# Autodesk Inventor assembly: GE-17025_ASM_174_ASM
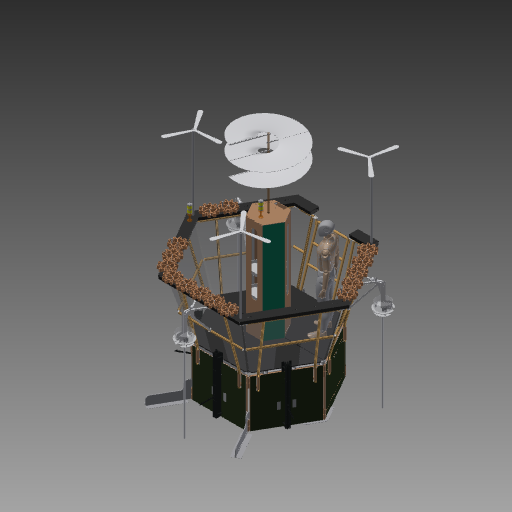
[picture p0: Inventor's stored thumbnail of the model, 512x512]
Saved by Autodesk Inventor 2017.1 (Build 211199000, 199)
## iProperties
Created: 2016-12-16
Part Number: GE-17025_ASM_174_ASM
Document SubType Name: Assembly
Designer: PhillipD
Author: PhillipD
Revision Number: 1LAST_VERSION
## Documents named in this file (25)
- D:\FIRST\FIRST KOP 2017\FRC 2017 Field\Parts\GE-17025_ASM_174_ASM.iam
- D:\FIRST\FIRST KOP 2017\FRC 2017 Field\Parts\GE-17026_ASM_28_ASM.iam
- D:\FIRST\FIRST KOP 2017\FRC 2017 Field\Parts\GE-17033_ASM_16_ASM.iam
- D:\FIRST\FIRST KOP 2017\FRC 2017 Field\Parts\GE-17034_6.ipt
- D:\FIRST\FIRST KOP 2017\FRC 2017 Field\Parts\GE-17044_ASM_20_ASM.iam
- D:\FIRST\FIRST KOP 2017\FRC 2017 Field\Parts\GE-17079_ASM_12_ASM.iam
- D:\FIRST\FIRST KOP 2017\FRC 2017 Field\Parts\AS2_ROPE_6.ipt
- D:\FIRST\FIRST KOP 2017\FRC 2017 Field\Parts\GE-17046_ASM_34_ASM.iam
- D:\FIRST\FIRST KOP 2017\FRC 2017 Field\Parts\GE-17075_ASM_7_ASM.iam
- D:\FIRST\FIRST KOP 2017\FRC 2017 Field\Parts\GE-17085_8.ipt
- D:\FIRST\FIRST KOP 2017\FRC 2017 Field\Parts\GE-17088_ASM_44_ASM.iam
- D:\FIRST\FIRST KOP 2017\FRC 2017 Field\Parts\GE-17092_3.ipt
- D:\FIRST\FIRST KOP 2017\FRC 2017 Field\Parts\GE-17098_14.ipt
- D:\FIRST\FIRST KOP 2017\FRC 2017 Field\Parts\GE-17099_6.ipt
- D:\FIRST\FIRST KOP 2017\FRC 2017 Field\Parts\GE-17069_ASM_14_ASM.iam
- D:\FIRST\FIRST KOP 2017\FRC 2017 Field\Parts\GE-17070_11.ipt
- D:\FIRST\FIRST KOP 2017\FRC 2017 Field\Parts\GE-17071_ASM_15_ASM.iam
- D:\FIRST\FIRST KOP 2017\FRC 2017 Field\Parts\GE-17072_ASM_9_ASM.iam
- D:\FIRST\FIRST KOP 2017\FRC 2017 Field\Parts\GE-17101_ASM_13_ASM.iam
- D:\FIRST\FIRST KOP 2017\FRC 2017 Field\Parts\LIGHT_ASM_ASM_3_ASM.iam
- D:\FIRST\FIRST KOP 2017\FRC 2017 Field\Parts\TOUCHPAD_ASSEMBLY_V3_ASM_ASM_2_ASM.iam
- D:\FIRST\FIRST KOP 2017\FRC 2017 Field\Parts\GE-17025-01_1.ipt
- D:\FIRST\FIRST KOP 2017\FRC 2017 Field\Parts\FUEL_TANK_ASM_1_ASM.iam
- D:\FIRST\FIRST KOP 2017\FRC 2017 Field\Parts\DA_VINCI_PROP_ASM_1_ASM.iam
- D:\FIRST\FIRST KOP 2017\FRC 2017 Field\Parts\JARDE_DUMMY_ASM_3_ASM.iam
## Components (70 placed, 70 different names)
1. GE-17026_ASM_28_ASM_1105 [sub-assembly]
2. GE-17033_ASM_16_ASM_1117 [sub-assembly]
3. GE-17033_ASM_16_ASM_1118 [sub-assembly]
4. GE-17034_6_1119 — Flush:2, Flush:4, Mate:2, Mate:7, Mate:8, Mate:9
5. GE-17034_6_1120 — Flush:3, Flush:5, Flush:8, Flush:9
6. GE-17044_ASM_20_ASM_1130 [sub-assembly] — Tangent:6
7. GE-17044_ASM_20_ASM_1131 [sub-assembly] — Tangent:8
8. GE-17044_ASM_20_ASM_1132 [sub-assembly]
9. GE-17044_ASM_20_ASM_1133 [sub-assembly]
10. GE-17044_ASM_20_ASM_1134 [sub-assembly] — Tangent:7
11. GE-17079_ASM_12_ASM_1151 [sub-assembly]
12. GE-17079_ASM_12_ASM_1152 [sub-assembly] — Mate:10, Mate:11
13. GE-17079_ASM_12_ASM_1153 [sub-assembly]
14. JARDE_DUMMY_ASM_3_ASM_1154 [sub-assembly]
15. AS2_ROPE_6_1155
16. AS2_ROPE_6_1156
17. AS2_ROPE_6_1157
18. GE-17046_ASM_34_ASM_1213 [sub-assembly]
19. GE-17046_ASM_34_ASM_1214 [sub-assembly]
20. GE-17046_ASM_34_ASM_1215 [sub-assembly]
21. GE-17075_ASM_7_ASM_1222 [sub-assembly]
22. GE-17075_ASM_7_ASM_1223 [sub-assembly]
23. GE-17085_8_1224
24. GE-17085_8_1225
25. GE-17085_8_1226
26. GE-17085_8_1227
27. GE-17085_8_1228
28. GE-17085_8_1229
29. GE-17088_ASM_44_ASM_1277 [sub-assembly] — Insert:1, Insert:2, Insert:3, Flush:5, Flush:6, Flush:7, Flush:8, Flush:9, Insert:4, Insert:5, Mate:4, Mate:5, Insert:6, Insert:7, Insert:8, Insert:9, Insert:10, Insert:11, Insert:12, Insert:13, Tangent:3, Insert:14, Insert:15, Insert:16, Insert:17, Insert:18, Tangent:4, Drive Me Gears 1, Tangent:9, Drive Me Gears 2
30. GE-17092_3_1278 — Insert:3
31. GE-17092_3_1279 — Insert:1
32. GE-17092_3_1280 — Insert:2
33. GE-17098_14_1281 — Mate:9, Tangent:8
34. GE-17098_14_1282 — Mate:7, Tangent:6
35. GE-17098_14_1283 — Mate:8, Tangent:7
36. GE-17099_6_1284
37. GE-17099_6_1285
38. GE-17069_ASM_14_ASM_1292 [sub-assembly]
39. GE-17070_11_1293
40. GE-17070_11_1294
41. GE-17071_ASM_15_ASM_1304 [sub-assembly]
42. GE-17072_ASM_9_ASM_1310 [sub-assembly]
43. GE-17101_ASM_13_ASM_1313 [sub-assembly] — Insert:4, Rotation:1, Align Gears 1
44. GE-17101_ASM_13_ASM_1314 [sub-assembly] — Insert:5, Rotation:1, Align Gears 1, Drive Me Gears 1, Tangent:9
45. GE-17101_ASM_13_ASM_1315 [sub-assembly] — Insert:6, Tangent:3, Align Gears 2a, Drive Me Gears 2, Rotation:2
46. GE-17101_ASM_13_ASM_1316 [sub-assembly] — Insert:7, Align Gears 2a, Align Gears 2b, Rotation:2, Rotation:3
47. GE-17101_ASM_13_ASM_1317 [sub-assembly] — Insert:8, Align Gears 2b, Align Gears 2c, Rotation:3, Rotation:4
48. GE-17101_ASM_13_ASM_1318 [sub-assembly] — Insert:9, Align Gears 2d, Align Gears 2c, Rotation:4, Rotation:5
49. GE-17101_ASM_13_ASM_1319 [sub-assembly] — Insert:10, Align Gears 2e, Align Gears 2d, Rotation:5, Rotation:8
50. GE-17101_ASM_13_ASM_1320 [sub-assembly] — Insert:11, Align Gears 2f, Align Gears 2e, Rotation:6, Rotation:8
51. GE-17101_ASM_13_ASM_1321 [sub-assembly] — Insert:12, Align Gears 2g, Align Gears 2f, Rotation:6, Rotation:7
52. GE-17101_ASM_13_ASM_1322 [sub-assembly] — Insert:13, Align Gears 2g, Rotation:7
53. GE-17101_ASM_13_ASM_1323 [sub-assembly] — Insert:14, Tangent:4
54. GE-17101_ASM_13_ASM_1324 [sub-assembly] — Insert:15
55. GE-17101_ASM_13_ASM_1325 [sub-assembly] — Insert:16
56. GE-17101_ASM_13_ASM_1326 [sub-assembly] — Insert:17
57. GE-17101_ASM_13_ASM_1327 [sub-assembly] — Insert:18
58. LIGHT_ASM_ASM_3_ASM_1335 [sub-assembly] — Mate:4, Mate:5
59. LIGHT_ASM_ASM_3_ASM_1336 [sub-assembly]
60. TOUCHPAD_ASSEMBLY_V3_ASM_ASM_2_ASM_1376 [sub-assembly] — Flush:10, Mate:10, Mate:11
61. TOUCHPAD_ASSEMBLY_V3_ASM_ASM_2_ASM_1377 [sub-assembly] — Flush:10
62. TOUCHPAD_ASSEMBLY_V3_ASM_ASM_2_ASM_1378 [sub-assembly]
63. GE-17025-01_1_1379
64. GE-17025-01_1_1380
65. GE-17025-01_1_1381
66. GE-17025-01_1_1382
67. GE-17025-01_1_1383
68. GE-17025-01_1_1384
69. FUEL_TANK_ASM_1_ASM_1416 [sub-assembly] — Mate:1, Flush:1, Flush:2, Flush:3, Flush:4, Mate:2, Flush:6, Flush:7
70. DA_VINCI_PROP_ASM_1_ASM_1424 [sub-assembly] — Mate:1, Flush:1
## Relationships (61: Insert 18, Mate 16, Flush 10, RelateRotation 8, Tangent 6, Angle 3)
- Insert:1: GE-17088_ASM_44_ASM_1277 ↔ GE-17092_3_1279
- Insert:2: GE-17088_ASM_44_ASM_1277 ↔ GE-17092_3_1280
- Insert:3: GE-17088_ASM_44_ASM_1277 ↔ GE-17092_3_1278
- Mate:1: FUEL_TANK_ASM_1_ASM_1416 ↔ DA_VINCI_PROP_ASM_1_ASM_1424
- Flush:1 (-1266.825 mm): FUEL_TANK_ASM_1_ASM_1416 ↔ DA_VINCI_PROP_ASM_1_ASM_1424
- Flush:2 (635 mm): GE-17034_6_1119 ↔ FUEL_TANK_ASM_1_ASM_1416
- Flush:3 (635.0254 mm): GE-17034_6_1120 ↔ FUEL_TANK_ASM_1_ASM_1416
- Flush:4 (635 mm): GE-17034_6_1119 ↔ FUEL_TANK_ASM_1_ASM_1416
- Mate:2: GE-17034_6_1119 ↔ FUEL_TANK_ASM_1_ASM_1416
- Flush:5 (-1107.2876 mm): GE-17034_6_1120 ↔ GE-17088_ASM_44_ASM_1277
- Flush:6 (1015.0602 mm): GE-17088_ASM_44_ASM_1277 ↔ FUEL_TANK_ASM_1_ASM_1416
- Flush:7 (1014.603 mm): GE-17088_ASM_44_ASM_1277 ↔ FUEL_TANK_ASM_1_ASM_1416
- Flush:8 (-1107.2876 mm): GE-17034_6_1120 ↔ GE-17088_ASM_44_ASM_1277
- Flush:9 (-1107.2876 mm): GE-17034_6_1120 ↔ GE-17088_ASM_44_ASM_1277
- Insert:4: GE-17088_ASM_44_ASM_1277 ↔ GE-17101_ASM_13_ASM_1313
- Insert:5: GE-17088_ASM_44_ASM_1277 ↔ GE-17101_ASM_13_ASM_1314
- Rotation:1 [RelateRotation] (1 ul): GE-17101_ASM_13_ASM_1313 ↔ GE-17101_ASM_13_ASM_1314
- Mate:4: GE-17088_ASM_44_ASM_1277 ↔ LIGHT_ASM_ASM_3_ASM_1335
- Mate:5: GE-17088_ASM_44_ASM_1277 ↔ LIGHT_ASM_ASM_3_ASM_1335
- Insert:6: GE-17088_ASM_44_ASM_1277 ↔ GE-17101_ASM_13_ASM_1315
- Insert:7: GE-17088_ASM_44_ASM_1277 ↔ GE-17101_ASM_13_ASM_1316
- Insert:8: GE-17088_ASM_44_ASM_1277 ↔ GE-17101_ASM_13_ASM_1317
- Insert:9: GE-17088_ASM_44_ASM_1277 ↔ GE-17101_ASM_13_ASM_1318
- Insert:10: GE-17088_ASM_44_ASM_1277 ↔ GE-17101_ASM_13_ASM_1319
- Insert:11: GE-17088_ASM_44_ASM_1277 ↔ GE-17101_ASM_13_ASM_1320
- Insert:12: GE-17088_ASM_44_ASM_1277 ↔ GE-17101_ASM_13_ASM_1321
- Insert:13: GE-17088_ASM_44_ASM_1277 ↔ GE-17101_ASM_13_ASM_1322
- Tangent:3: GE-17088_ASM_44_ASM_1277 ↔ GE-17101_ASM_13_ASM_1315
- Insert:14: GE-17088_ASM_44_ASM_1277 ↔ GE-17101_ASM_13_ASM_1323
- Insert:15: GE-17088_ASM_44_ASM_1277 ↔ GE-17101_ASM_13_ASM_1324
- Insert:16: GE-17088_ASM_44_ASM_1277 ↔ GE-17101_ASM_13_ASM_1325
- Insert:17: GE-17088_ASM_44_ASM_1277 ↔ GE-17101_ASM_13_ASM_1326
- Insert:18: GE-17088_ASM_44_ASM_1277 ↔ GE-17101_ASM_13_ASM_1327
- Tangent:4: GE-17088_ASM_44_ASM_1277 ↔ GE-17101_ASM_13_ASM_1323
- Align Gears 1 [Mate]: GE-17101_ASM_13_ASM_1313 ↔ GE-17101_ASM_13_ASM_1314
- Drive Me Gears 1 [Angle] (0 deg): GE-17088_ASM_44_ASM_1277 ↔ GE-17101_ASM_13_ASM_1314
- Mate:7: GE-17034_6_1119 ↔ GE-17098_14_1282
- Tangent:6: GE-17044_ASM_20_ASM_1130 ↔ GE-17098_14_1282
- Mate:8: GE-17034_6_1119 ↔ GE-17098_14_1283
- Tangent:7: GE-17044_ASM_20_ASM_1134 ↔ GE-17098_14_1283
- Mate:9: GE-17034_6_1119 ↔ GE-17098_14_1281
- Tangent:8: GE-17044_ASM_20_ASM_1131 ↔ GE-17098_14_1281
- Flush:10: TOUCHPAD_ASSEMBLY_V3_ASM_ASM_2_ASM_1376 ↔ TOUCHPAD_ASSEMBLY_V3_ASM_ASM_2_ASM_1377
- Mate:10: GE-17079_ASM_12_ASM_1152 ↔ TOUCHPAD_ASSEMBLY_V3_ASM_ASM_2_ASM_1376
- Mate:11: GE-17079_ASM_12_ASM_1152 ↔ TOUCHPAD_ASSEMBLY_V3_ASM_ASM_2_ASM_1376
- Tangent:9: GE-17088_ASM_44_ASM_1277 ↔ GE-17101_ASM_13_ASM_1314
- Align Gears 2a [Mate]: GE-17101_ASM_13_ASM_1315 ↔ GE-17101_ASM_13_ASM_1316
- Align Gears 2b [Mate]: GE-17101_ASM_13_ASM_1316 ↔ GE-17101_ASM_13_ASM_1317
- Drive Me Gears 2 [Angle] (0 deg): GE-17088_ASM_44_ASM_1277 ↔ GE-17101_ASM_13_ASM_1315
- Rotation:2 [RelateRotation] (1 ul): GE-17101_ASM_13_ASM_1315 ↔ GE-17101_ASM_13_ASM_1316
- Align Gears 2g [Mate]: GE-17101_ASM_13_ASM_1321 ↔ GE-17101_ASM_13_ASM_1322
- Align Gears 2f [Mate]: GE-17101_ASM_13_ASM_1320 ↔ GE-17101_ASM_13_ASM_1321
- Align Gears 2e [Mate]: GE-17101_ASM_13_ASM_1319 ↔ GE-17101_ASM_13_ASM_1320
- Align Gears 2d [Mate]: GE-17101_ASM_13_ASM_1318 ↔ GE-17101_ASM_13_ASM_1319
- Align Gears 2c [Angle] (0 deg): GE-17101_ASM_13_ASM_1317 ↔ GE-17101_ASM_13_ASM_1318
- Rotation:3 [RelateRotation] (1 ul): GE-17101_ASM_13_ASM_1316 ↔ GE-17101_ASM_13_ASM_1317
- Rotation:4 [RelateRotation] (1 ul): GE-17101_ASM_13_ASM_1317 ↔ GE-17101_ASM_13_ASM_1318
- Rotation:5 [RelateRotation] (1 ul): GE-17101_ASM_13_ASM_1318 ↔ GE-17101_ASM_13_ASM_1319
- Rotation:6 [RelateRotation] (1 ul): GE-17101_ASM_13_ASM_1320 ↔ GE-17101_ASM_13_ASM_1321
- Rotation:7 [RelateRotation] (1 ul): GE-17101_ASM_13_ASM_1321 ↔ GE-17101_ASM_13_ASM_1322
- Rotation:8 [RelateRotation] (1 ul): GE-17101_ASM_13_ASM_1319 ↔ GE-17101_ASM_13_ASM_1320
